# Autodesk Inventor assembly: FE-000 Rectangle Field
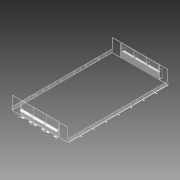
[picture p0: Inventor's stored thumbnail of the model, 180x180]
Saved by Autodesk Inventor 2021 (Build 250183000, 183)
## iProperties
Created: 2021-01-11
Part Number: FE-000 Rectangle Field
Document SubType Name: Assembly
## Documents named in this file (5)
- D:\FIRST\Design\FRC Fields\Generic Field Base\Configurable Field.iam
- D:\FIRST\Design\FRC Fields\Generic Field Base\FE-100 Side Wall\FE-100 Side Wall.iam
- D:\FIRST\Design\FRC Fields\Generic Field Base\FE-200 Driver Station\FE-210 Main Stall\FE-210 Main Stall.ipt
- D:\FIRST\Design\FRC Fields\Generic Field Base\FE-200 Driver Station\FE-220 Connectors\FE-220 Connectors.ipt
- D:\FIRST\Design\FRC Fields\Generic Field Base\FE-200 Driver Station\FE-230 Doors\FE-230 Doorway.ipt
## Components (20 placed, 4 different names)
1. FE-100 Side Wall:1 [sub-assembly] — Flush:1, Flush:2, Symmetry:1, Mate:1, Flush:3, Flush:7, Mate:7
2. FE-100 Side Wall:2 [sub-assembly] — Flush:1, Flush:2, Symmetry:1, Mate:9
3. FE-230 Doorway:1 — Flush:8, Flush:9, Mate:6, Flush:10, Symmetry:3
4. FE-230 Doorway:2 — Flush:8, Flush:9, Flush:11, Symmetry:3, Mate:7
5. FE-230 Doorway:3 — Mate:8, Mate:9, Flush:12, Symmetry:4, Flush:14
6. FE-230 Doorway:4 — Flush:13, Symmetry:4, Flush:14
7. FE-210 Main Stall:2 — Flush:4, Flush:5, Symmetry:2, Mate:2, Mate:4, Tangent:1, Flush:7, Flush:11
8. FE-210 Main Stall:1 — Flush:4, Flush:5, Symmetry:2, Mate:3, Mate:5, Flush:10
9. FE-210 Main Stall:3
10. FE-210 Main Stall:4
11. FE-210 Main Stall:5
12. FE-210 Main Stall:6
13. FE-220 Connectors:1 — Mate:2, Flush:6, Mate:4, Tangent:1
14. FE-220 Connectors:2 — Mate:3, Flush:6, Mate:5, Mate:6
15. FE-220 Connectors:3
16. FE-220 Connectors:4
17. FE-220 Connectors:5
18. FE-220 Connectors:6
19. FE-220 Connectors:7 — Mate:8, Flush:12
20. FE-220 Connectors:8 — Flush:13
## Component patterns: (3 elements, first: FE-210 Main Stall:2 + FE-210 Main Stall:1), (4 elements, first: FE-220 Connectors:1 + FE-220 Connectors:2)
## Relationships (28: Flush 14, Mate 9, Symmetry 4, Tangent 1)
- Flush:1: FE-100 Side Wall:1 ↔ FE-100 Side Wall:2
- Flush:2: FE-100 Side Wall:1 ↔ FE-100 Side Wall:2
- Symmetry:1: FE-100 Side Wall:1 ↔ FE-100 Side Wall:2
- Mate:1: FE-100 Side Wall:1
- Flush:3: FE-100 Side Wall:1
- Flush:4: FE-210 Main Stall:2 ↔ FE-210 Main Stall:1
- Flush:5: FE-210 Main Stall:2 ↔ FE-210 Main Stall:1
- Symmetry:2: FE-210 Main Stall:2 ↔ FE-210 Main Stall:1
- Mate:2: FE-210 Main Stall:2 ↔ FE-220 Connectors:1
- Mate:3: FE-210 Main Stall:1 ↔ FE-220 Connectors:2
- Flush:6: FE-220 Connectors:1 ↔ FE-220 Connectors:2
- Mate:4: FE-210 Main Stall:2 ↔ FE-220 Connectors:1
- Mate:5: FE-210 Main Stall:1 ↔ FE-220 Connectors:2
- Tangent:1: FE-210 Main Stall:2 ↔ FE-220 Connectors:1
- Flush:7: FE-100 Side Wall:1 ↔ FE-210 Main Stall:2
- Flush:8: FE-230 Doorway:1 ↔ FE-230 Doorway:2
- Flush:9: FE-230 Doorway:1 ↔ FE-230 Doorway:2
- Mate:6: FE-230 Doorway:1 ↔ FE-220 Connectors:2
- Flush:10: FE-230 Doorway:1 ↔ FE-210 Main Stall:1
- Flush:11: FE-230 Doorway:2 ↔ FE-210 Main Stall:2
- Symmetry:3: FE-230 Doorway:1 ↔ FE-230 Doorway:2
- Mate:7: FE-100 Side Wall:1 ↔ FE-230 Doorway:2
- Mate:8: FE-230 Doorway:3 ↔ FE-220 Connectors:7
- Mate:9: FE-100 Side Wall:2 ↔ FE-230 Doorway:3
- Flush:12: FE-230 Doorway:3 ↔ FE-220 Connectors:7
- Flush:13: FE-230 Doorway:4 ↔ FE-220 Connectors:8
- Symmetry:4: FE-230 Doorway:3 ↔ FE-230 Doorway:4
- Flush:14: FE-230 Doorway:3 ↔ FE-230 Doorway:4
